# Autodesk Inventor assembly: VESA mounting
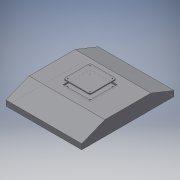
[picture p0: Inventor's stored thumbnail of the model, 180x180]
Saved by Autodesk Inventor 2016 (Build 200138000, 138)
## iProperties
Created: 2017-11-15
Part Number: VESA mounting
Document SubType Name: Assembly
Designer: student
Author: student
## Documents named in this file (3)
- C:\Users\student\Documents\Aaron's Folder\VESA mounting.iam
- C:\Users\student\Documents\Aaron's Folder\monitor (for assembly).ipt
- C:\Users\student\Documents\Aaron's Folder\VESA mount.ipt
## Components (2 placed, 2 different names)
1. monitor (for assembly):1 — Rigid:1
2. VESA mount:1 — Rigid:1
## Relationships (1: WeldJoint 1)
- Rigid:1 [WeldJoint] (25.4 mm): monitor (for assembly):1 ↔ VESA mount:1
